(part 1 of 3)
# Autodesk Inventor assembly: FirstIntakes
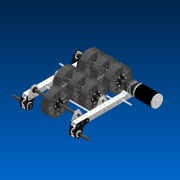
[picture p0: Inventor's stored thumbnail of the model, 180x180]
Saved by Autodesk Inventor 2022 (Build 260153000, 153)
## iProperties
Created: 2022-01-09
Part Number: FirstIntakes
Document SubType Name: Assembly
Designer: omard
Author: omard
## Documents named in this file (30)
- C:\Users\score_nygvs6w\OneDrive - Auburn University\BasketBall Shooting Robot\FirstIntakes.iam
- C:\Users\score_nygvs6w\OneDrive - Auburn University\BasketBall Shooting Robot\VEX Parts\VersaFrame Side Bearing Gusset (217-3553).ipt
- C:\Users\score_nygvs6w\OneDrive - Auburn University\BasketBall Shooting Robot\VEX Parts\13.75mm (1_2 ThunderHex ID) x 1.125 OD x 0.313 WD (Flanged Bearing) (217-4006).ipt
- C:\Users\score_nygvs6w\OneDrive - Auburn University\BasketBall Shooting Robot\VEX Parts\5 Straight Flex Wheel (60A) (217-6455).ipt
- C:\Users\score_nygvs6w\OneDrive - Auburn University\BasketBall Shooting Robot\VEX Parts\1_2” Hex Bore Plastic VersaHub v2 (217-8079).iam
- C:\Users\score_nygvs6w\OneDrive - Auburn University\BasketBall Shooting Robot\VEX Parts\24T x 9mm Wide Double Flange Aluminum Pulley (HTD 5mm, 1_2” Hex Bore) (217-3227).ipt
- C:\Users\score_nygvs6w\OneDrive - Auburn University\BasketBall Shooting Robot\VEX Parts\#8-32 x 2.000 Star Drive Screw (276-8015).ipt
- C:\Users\score_nygvs6w\OneDrive - Auburn University\BasketBall Shooting Robot\VEX Parts\#8-32 Nylock Nut (275-1027).ipt
- C:\Users\score_nygvs6w\OneDrive - Auburn University\BasketBall Shooting Robot\VEX Parts\1_4 Acetal Spacer - 1_2 Hex (217-2758).ipt
- C:\Users\score_nygvs6w\OneDrive - Auburn University\BasketBall Shooting Robot\VEX Parts\1_2 Acetal Spacer - 1_2 Hex (217-2758).ipt
- C:\Users\score_nygvs6w\OneDrive - Auburn University\BasketBall Shooting Robot\VEX Parts\80T x 9mm Wide Timing Belt (HTD 5mm)(217-3456).ipt
- C:\Users\score_nygvs6w\OneDrive - Auburn University\BasketBall Shooting Robot\VEX Parts\Clamping Shaft Collar - 1_2 Hex ID (217-2737).ipt
- C:\Users\score_nygvs6w\OneDrive - Auburn University\BasketBall Shooting Robot\VEX Parts\1_16 Acetal Spacer - 1_2 Hex (217-2758).ipt
- C:\Users\score_nygvs6w\OneDrive - Auburn University\BasketBall Shooting Robot\VEX Parts\#8-32 x 1.500 Star Drive Screw (276-4998).ipt
- C:\Users\score_nygvs6w\OneDrive - Auburn University\BasketBall Shooting Robot\Intake Joint Holder Using 1__16 Gray Tinted Polycarbonate Sheet (36 x 72) (217-6627).ipt
- C:\Users\score_nygvs6w\OneDrive - Auburn University\BasketBall Shooting Robot\VEX Parts\1.00 Standoff (275-1016).ipt
- C:\Users\score_nygvs6w\OneDrive - Auburn University\BasketBall Shooting Robot\VEX Parts\#8-32 x 0.500 Star Drive Screw (276-4992).ipt
- C:\Users\score_nygvs6w\OneDrive - Auburn University\BasketBall Shooting Robot\VEX Parts\1_8 Acetal Spacer - 1_2 Hex (217-2758).ipt
- C:\Users\score_nygvs6w\OneDrive - Auburn University\BasketBall Shooting Robot\VEX Parts\VersaPlanetary v2 One Stage Universal Output.iam
- C:\Users\score_nygvs6w\OneDrive - Auburn University\BasketBall Shooting Robot\VEX Parts\Special Cut\Intake VersaFrame VersaPlanetary Side Mount Modified (217-4239).ipt
- C:\Users\score_nygvs6w\OneDrive - Auburn University\BasketBall Shooting Robot\Intake Motor Holder Using 1__16 Gray Tinted Polycarbonate Sheet (36 x 72) (217-6627).ipt
- C:\Users\score_nygvs6w\OneDrive - Auburn University\BasketBall Shooting Robot\VEX Parts\Falcon 500, Powered by Talon FX (217-6515).iam
- C:\Users\score_nygvs6w\OneDrive - Auburn University\BasketBall Shooting Robot\VEX Parts\Special Cut\1 x 1 x 0.040 x 14 Intake Pre-Drilled VersaFrame Aluminum Tube Stock Cut Modified (217-3426).ipt
- C:\Users\score_nygvs6w\OneDrive - Auburn University\BasketBall Shooting Robot\VEX Parts\1_2 Hex x 0.201 x 10.5 ID ThunderHex Stock Cut (217-4017).ipt
- C:\Users\score_nygvs6w\OneDrive - Auburn University\BasketBall Shooting Robot\VEX Parts\1_2 Hex x 0.201 x 11 ID ThunderHex Stock Cut (217-4017).ipt
- C:\Users\score_nygvs6w\OneDrive - Auburn University\BasketBall Shooting Robot\VEX Parts\1_2 Hex x 0.201 x 4 ID ThunderHex Stock Cut (217-4017).ipt
- C:\Users\score_nygvs6w\OneDrive - Auburn University\BasketBall Shooting Robot\VEX Parts\5.00 Standoff  (275-1022).ipt
- C:\Users\score_nygvs6w\OneDrive - Auburn University\BasketBall Shooting Robot\VEX Parts\#8-32 x 1.000 Star Drive Coupler (276-4988).ipt
- C:\Users\score_nygvs6w\OneDrive - Auburn University\BasketBall Shooting Robot\VEX Parts\2.00 Standoff  (275-1018).ipt
- C:\Users\score_nygvs6w\OneDrive - Auburn University\BasketBall Shooting Robot\VEX Parts\CIM Motor (217-2000).ipt
## Components (233 placed, 29 different names)
1. VersaFrame Side Bearing Gusset (217-3553):2 — Mate:8, Mate:9, Mate:10, Mate:12, Mate:15, Mate:521, Mate:522
2. VersaFrame Side Bearing Gusset (217-3553):3 — Mate:1, Mate:2, Mate:3, Angle:1, Mate:13, Mate:14, Mate:523, Mate:524, Mate:525, Mate:636
3. 1 x 1 x 0.040 x 14 Intake Pre-Drilled VersaFrame Aluminum Tube Stock Cut Modified (217-3426):1 — Mate:1, Mate:2, Mate:3, Mate:8, Mate:9, Mate:10, Angle:1, Angle:2, Angle:3, Angle:20, Angle:133, Angle:134, Angle:135, Angle:136, Mate:494, Mate:495, Mate:496, Mate:497, Mate:498, Mate:499, Mate:500, Mate:501, Mate:505, Mate:506, Angle:203, Angle:204, Angle:205, Angle:206, Angle:207, Angle:208, Angle:209, Angle:210, Angle:211, Angle:212, Angle:213, Angle:214, Angle:215, Angle:216, Angle:217, Angle:218, Angle:258, Mate:630, Mate:631, Mate:632, Mate:633, Mate:634, Mate:635, Angle:262, Angle:263, Angle:264, Angle:265, Angle:266, Angle:268, Angle:274, Mate:699, Mate:700, Mate:701, Mate:702, Mate:703, Mate:704, Angle:279, Angle:280, Angle:281, Angle:282, Angle:283, Angle:284, Angle:285, Angle:286, Angle:287, Angle:288, Angle:289, Angle:290, Angle:291, Angle:292, Angle:293, Angle:294, Angle:295, Angle:296, Angle:297, Angle:298, Angle:299, Angle:300, Angle:301, Angle:302, Angle:303, Angle:304, Angle:305, Angle:306, Angle:307, Angle:308, Angle:309, Angle:310, Angle:311, Angle:312, Angle:313, Angle:314, Angle:317, Flush:563, Mate:742, Mate:743, Mate:744, Mate:745, Angle:330, Angle:331, Angle:335, Mate:752, Mate:753, Mate:754, Mate:757, Angle:337
4. 13.75mm (1_2 ThunderHex ID) x 1.125 OD x 0.313 WD (Flanged Bearing) (217-4006):1 — Mate:13, Mate:14, Mate:19, Angle:2, Mate:629, Mate:712, Flush:562
5. 13.75mm (1_2 ThunderHex ID) x 1.125 OD x 0.313 WD (Flanged Bearing) (217-4006):2 — Mate:12, Mate:15, Angle:3, Mate:448, Mate:526, Mate:713, Flush:561
6. 5 Straight Flex Wheel (60A) (217-6455):3 — Mate:19, Mate:22, Mate:23, Mate:28, Mate:31, Mate:34, Mate:37, Flush:2, Mate:455, Mate:558, Flush:560, Flush:14, Mate:610
7. 1_2” Hex Bore Plastic VersaHub v2 (217-8079):1 [sub-assembly] — Mate:31, Mate:34, Mate:37, Mate:90, Mate:93, Mate:94, Mate:95, Mate:96, Mate:97, Mate:98, Mate:99, Mate:100, Mate:101, Mate:102, Mate:103, Mate:104, Mate:117, Angle:35, Mate:118
8. 1_2” Hex Bore Plastic VersaHub v2 (217-8079):4 [sub-assembly] — Mate:22, Mate:23, Mate:28, Mate:111, Mate:112, Mate:113, Mate:114, Mate:115, Mate:116, Angle:23, Angle:24, Angle:25, Angle:26, Angle:27, Angle:28, Angle:185, Angle:186, Mate:467, Mate:468
9. 24T x 9mm Wide Double Flange Aluminum Pulley (HTD 5mm, 1_2” Hex Bore) (217-3227):3 — Mate:90, Angle:20, Angle:29, Angle:30, Angle:31, Angle:32, Angle:33, Angle:34, Angle:36, Mate:119, Flush:5, Mate:470, Mate:471, Mate:472, Angle:188
10. 1_4 Acetal Spacer - 1_2 Hex (217-2758):14 — Mate:117, Angle:35, Mate:118, Angle:36, Mate:119
11. 5 Straight Flex Wheel (60A) (217-6455):4 — Mate:406, Mate:407, Flush:1, Flush:2, Mate:448, Mate:477
12. 1_2” Hex Bore Plastic VersaHub v2 (217-8079):5 [sub-assembly]
13. 1_2” Hex Bore Plastic VersaHub v2 (217-8079):6 [sub-assembly] — Angle:219, Angle:221, Angle:222, Angle:223, Angle:224, Angle:220, Mate:547, Mate:548, Mate:550, Mate:551, Mate:552, Mate:553
14. 24T x 9mm Wide Double Flange Aluminum Pulley (HTD 5mm, 1_2” Hex Bore) (217-3227):5 — Mate:476
15. 1_4 Acetal Spacer - 1_2 Hex (217-2758):12 — Mate:463
16. 1_4 Acetal Spacer - 1_2 Hex (217-2758):11
17. 24T x 9mm Wide Double Flange Aluminum Pulley (HTD 5mm, 1_2” Hex Bore) (217-3227):6 — Angle:134, Mate:452, Flush:6
18. 5 Straight Flex Wheel (60A) (217-6455):5 — Mate:410, Mate:444, Flush:1
19. 1_2” Hex Bore Plastic VersaHub v2 (217-8079):7 [sub-assembly]
20. 1_2” Hex Bore Plastic VersaHub v2 (217-8079):8 [sub-assembly] — Angle:225, Angle:226, Angle:227, Angle:228, Angle:229, Angle:230, Mate:541, Mate:542, Mate:543, Mate:544, Mate:545, Mate:546
21. 1_2 Acetal Spacer - 1_2 Hex (217-2758):4 — Mate:487
22. 1_4 Acetal Spacer - 1_2 Hex (217-2758):8
23. 24T x 9mm Wide Double Flange Aluminum Pulley (HTD 5mm, 1_2” Hex Bore) (217-3227):8 — Angle:133, Angle:139, Angle:140, Tangent:1
24. 5 Straight Flex Wheel (60A) (217-6455):6 — Mate:410, Flush:4, Mate:456
25. 1_2” Hex Bore Plastic VersaHub v2 (217-8079):9 [sub-assembly]
26. 1_2” Hex Bore Plastic VersaHub v2 (217-8079):10 [sub-assembly] — Angle:232, Mate:556, Mate:557
27. 1_4 Acetal Spacer - 1_2 Hex (217-2758):9
28. 5 Straight Flex Wheel (60A) (217-6455):10 — Mate:406, Flush:11, Mate:477
29. 1_2” Hex Bore Plastic VersaHub v2 (217-8079):17 [sub-assembly] — Mate:346, Mate:347, Mate:462, Angle:181, Mate:474
30. 1_2” Hex Bore Plastic VersaHub v2 (217-8079):18 [sub-assembly] — Mate:475
31. 1_4 Acetal Spacer - 1_2 Hex (217-2758):13 — Angle:135, Mate:474, Mate:476
32. 5 Straight Flex Wheel (60A) (217-6455):11 — Mate:407, Flush:4, Mate:453, Mate:454
33. 1_2” Hex Bore Plastic VersaHub v2 (217-8079):19 [sub-assembly]
34. 1_2” Hex Bore Plastic VersaHub v2 (217-8079):20 [sub-assembly] — Angle:136, Mate:464, Mate:465, Angle:183
35. 1_4 Acetal Spacer - 1_2 Hex (217-2758):10 — Mate:452
36. 5 Straight Flex Wheel (60A) (217-6455):12 — Mate:444, Flush:11
37. 1_2” Hex Bore Plastic VersaHub v2 (217-8079):21 [sub-assembly] — Angle:231, Mate:554, Mate:555
38. 1_2” Hex Bore Plastic VersaHub v2 (217-8079):22 [sub-assembly] — Mate:446, Angle:132, Mate:447
39. 1_2 Acetal Spacer - 1_2 Hex (217-2758):3 — Mate:446, Angle:132, Mate:447, Angle:139, Angle:140, Mate:486, Angle:199
40. 80T x 9mm Wide Timing Belt (HTD 5mm)(217-3456):1 — Mate:454, Mate:456, Flush:6, Tangent:1
41. 80T x 9mm Wide Timing Belt (HTD 5mm)(217-3456):2 — Mate:453, Mate:455, Flush:5
42. Clamping Shaft Collar - 1_2 Hex ID (217-2737):1 — Angle:258, Mate:682, Mate:711
43. Clamping Shaft Collar - 1_2 Hex ID (217-2737):3 — Mate:464, Mate:465, Angle:183, Angle:233
44. Clamping Shaft Collar - 1_2 Hex ID (217-2737):4 — Mate:462, Angle:181, Angle:182, Mate:475
45. Clamping Shaft Collar - 1_2 Hex ID (217-2737):6 — Angle:182, Mate:463, Mate:526, Angle:315
46. Clamping Shaft Collar - 1_2 Hex ID (217-2737):7 — Mate:470, Angle:189, Mate:629, Angle:316
47. Clamping Shaft Collar - 1_2 Hex ID (217-2737):9 — Angle:185, Angle:186, Mate:467, Mate:468
48. Clamping Shaft Collar - 1_2 Hex ID (217-2737):10 — Mate:471, Mate:472, Angle:188, Angle:189
49. 1_16 Acetal Spacer - 1_2 Hex (217-2758):2 — Mate:486, Angle:199, Mate:487
50. Clamping Shaft Collar - 1_2 Hex ID (217-2737):12 — Angle:231, Mate:554, Mate:555, Mate:682
51. Clamping Shaft Collar - 1_2 Hex ID (217-2737):11 — Angle:232, Mate:556, Mate:557, Angle:233, Mate:673
52. VersaFrame Side Bearing Gusset (217-3553):4 — Mate:621
53. VersaFrame Side Bearing Gusset (217-3553):5
54. 1 x 1 x 0.040 x 14 Intake Pre-Drilled VersaFrame Aluminum Tube Stock Cut Modified (217-3426):2 — Angle:255, Angle:257, Mate:614, Mate:615, Mate:616, Mate:618, Mate:619, Mate:620, Angle:259, Angle:260, Angle:261, Angle:267, Angle:273, Mate:666, Mate:667, Mate:668, Mate:719, Angle:328, Angle:329, Mate:738, Mate:739, Mate:740, Mate:741, Mate:746, Mate:747, Mate:748, Mate:749, Angle:332, Angle:333, Mate:750, Mate:751, Angle:334, Mate:755, Mate:756, Angle:336
55. 13.75mm (1_2 ThunderHex ID) x 1.125 OD x 0.313 WD (Flanged Bearing) (217-4006):5 — Mate:628
56. 13.75mm (1_2 ThunderHex ID) x 1.125 OD x 0.313 WD (Flanged Bearing) (217-4006):6 — Mate:610, Mate:611, Mate:617
57. Clamping Shaft Collar - 1_2 Hex ID (217-2737):14 — Angle:257, Mate:628
58. Clamping Shaft Collar - 1_2 Hex ID (217-2737):15 — Mate:611, Angle:255, Mate:617
59. Intake Joint Holder Using 1__16 Gray Tinted Polycarbonate Sheet (36 x 72) (217-6627):1 — Mate:584, Mate:585, Mate:583, Mate:614, Mate:615, Mate:616, Mate:622, Mate:623, Mate:626, Mate:627, Mate:650, Mate:651
60. Intake Joint Holder Using 1__16 Gray Tinted Polycarbonate Sheet (36 x 72) (217-6627):2 — Mate:618, Mate:619, Mate:620, Mate:621, Mate:625, Mate:652, Mate:653
61. Intake Joint Holder Using 1__16 Gray Tinted Polycarbonate Sheet (36 x 72) (217-6627):3 — Mate:630, Mate:631, Mate:632, Mate:636, Mate:641, Mate:643, Mate:645, Mate:647, Mate:649
62. Intake Joint Holder Using 1__16 Gray Tinted Polycarbonate Sheet (36 x 72) (217-6627):4 — Mate:633, Mate:634, Mate:635, Mate:637, Mate:638, Mate:639, Mate:642, Mate:644, Mate:646, Mate:648
63. 1.00 Standoff (275-1016):1 — Mate:622, Mate:623, Mate:624, Angle:261
64. 1.00 Standoff (275-1016):2 — Mate:643, Angle:264
65. 13.75mm (1_2 ThunderHex ID) x 1.125 OD x 0.313 WD (Flanged Bearing) (217-4006):7 — Mate:646, Mate:648, Angle:265, Mate:664, Mate:665, Mate:722, Mate:723
66. 13.75mm (1_2 ThunderHex ID) x 1.125 OD x 0.313 WD (Flanged Bearing) (217-4006):8 — Mate:652, Angle:268, Mate:653, Mate:724, Mate:725
67. 13.75mm (1_2 ThunderHex ID) x 1.125 OD x 0.313 WD (Flanged Bearing) (217-4006):9 — Mate:650, Mate:651, Angle:267, Mate:662, Mate:663, Mate:720, Mate:721
68. 13.75mm (1_2 ThunderHex ID) x 1.125 OD x 0.313 WD (Flanged Bearing) (217-4006):10 — Mate:647, Mate:649, Angle:266, Mate:726, Mate:727
69. 1_2 Acetal Spacer - 1_2 Hex (217-2758):5 — Mate:662, Mate:663, Angle:273, Angle:318
70. 1_4 Acetal Spacer - 1_2 Hex (217-2758):15
71. 1_8 Acetal Spacer - 1_2 Hex (217-2758):1 — Angle:320
72. 1_2 Acetal Spacer - 1_2 Hex (217-2758):6 — Angle:274, Angle:319, Angle:321
73. 1_4 Acetal Spacer - 1_2 Hex (217-2758):16
74. 1_8 Acetal Spacer - 1_2 Hex (217-2758):2 — Mate:664, Mate:665
75. Intake VersaFrame VersaPlanetary Side Mount Modified (217-4239):1 — Mate:666, Mate:667, Mate:668, Mate:669, Mate:670, Mate:671, Mate:590, Mate:674, Mate:675, Mate:676, Mate:677, Mate:678, Mate:679, Mate:680, Mate:681, Angle:275, Angle:276
76. VersaPlanetary v2 One Stage Universal Output:1 [sub-assembly] — Mate:669, Mate:670, Mate:671, Mate:673, Mate:714, Mate:715, Mate:716, Mate:718, Mate:758, Mate:759, Mate:760
77. Intake Motor Holder Using 1__16 Gray Tinted Polycarbonate Sheet (36 x 72) (217-6627):1 — Mate:701, Mate:702, Mate:703, Mate:708, Mate:709, Mate:710
78. Intake Motor Holder Using 1__16 Gray Tinted Polycarbonate Sheet (36 x 72) (217-6627):2 — Mate:699, Mate:700, Mate:704, Mate:705, Mate:706, Mate:707
79. 1.00 Standoff (275-1016):3 — Angle:279
80. 13.75mm (1_2 ThunderHex ID) x 1.125 OD x 0.313 WD (Flanged Bearing) (217-4006):11 — Angle:282, Mate:717
81. 13.75mm (1_2 ThunderHex ID) x 1.125 OD x 0.313 WD (Flanged Bearing) (217-4006):12 — Mate:711, Angle:283
82. 1_2 Acetal Spacer - 1_2 Hex (217-2758):7 — Angle:284
83. 1_4 Acetal Spacer - 1_2 Hex (217-2758):17
84. 1_8 Acetal Spacer - 1_2 Hex (217-2758):3
85. 1_2 Hex x 0.201 x 10.5 ID ThunderHex Stock Cut (217-4017):1 — Mate:712, Angle:316, Flush:562
86. 1_2 Hex x 0.201 x 10.5 ID ThunderHex Stock Cut (217-4017):2 — Mate:713, Angle:315, Flush:561
87. Falcon 500, Powered by Talon FX (217-6515):1 [sub-assembly] — Mate:714, Mate:715, Mate:716
88. 1_2 Hex x 0.201 x 11 ID ThunderHex Stock Cut (217-4017):1 — Mate:717, Angle:317, Mate:718
89. 1_2 Acetal Spacer - 1_2 Hex (217-2758):8 — Mate:720, Mate:721, Angle:318, Angle:322
90. 1_2 Acetal Spacer - 1_2 Hex (217-2758):9 — Angle:319, Mate:722, Mate:723
91. Clamping Shaft Collar - 1_2 Hex ID (217-2737):16 — Mate:724, Angle:320, Mate:725, Flush:565, Mate:728
92. Clamping Shaft Collar - 1_2 Hex ID (217-2737):17 — Angle:321, Mate:726, Mate:727, Angle:323, Flush:564, Mate:729
93. 1_2 Hex x 0.201 x 4 ID ThunderHex Stock Cut (217-4017):1 — Angle:322, Flush:565, Mate:728
94. 1_2 Hex x 0.201 x 4 ID ThunderHex Stock Cut (217-4017):2 — Angle:323, Flush:564, Mate:729
95. 5.00 Standoff  (275-1022):1 — Mate:730, Angle:324, Mate:732, Mate:733, Angle:329, Mate:738, Mate:740
96. 5.00 Standoff  (275-1022):2 — Mate:731, Angle:324, Mate:733, Angle:325
97. 5.00 Standoff  (275-1022):3 — Angle:328, Mate:739, Mate:741
98. 5.00 Standoff  (275-1022):4 — Angle:327
99. 2.00 Standoff  (275-1018):1 — Mate:750, Mate:751, Angle:334
100. 2.00 Standoff  (275-1018):2 — Angle:335, Mate:752, Mate:753
101. CIM Motor (217-2000):1 — Mate:758, Mate:759, Mate:760
102. #8-32 x 1.500 Star Drive Screw (276-4998):21 — Mate:755, Mate:756, Angle:336
103. #8-32 x 1.500 Star Drive Screw (276-4998):22 — Mate:754, Mate:757, Angle:337
104. #8-32 x 1.500 Star Drive Screw (276-4998):20 — Mate:743, Mate:745, Angle:330
105. #8-32 x 1.500 Star Drive Screw (276-4998):19 — Mate:742, Mate:744, Angle:331
106. #8-32 x 1.500 Star Drive Screw (276-4998):18 — Mate:746, Mate:749, Angle:332
107. #8-32 x 1.500 Star Drive Screw (276-4998):17 — Mate:747, Mate:748, Angle:333
108. #8-32 x 1.000 Star Drive Coupler (276-4988):1 — Mate:730, Mate:731, Mate:732, Angle:325
109. #8-32 x 1.000 Star Drive Coupler (276-4988):2 — Angle:327
110. #8-32 x 0.500 Star Drive Screw (276-4992):8 — Angle:281
111. #8-32 x 0.500 Star Drive Screw (276-4992):7 — Angle:280
112. #8-32 x 0.500 Star Drive Screw (276-4992):6 — Mate:678, Mate:681, Angle:276
113. #8-32 x 0.500 Star Drive Screw (276-4992):5 — Mate:679, Mate:680, Angle:275
114. #8-32 x 0.500 Star Drive Screw (276-4992):3 — Mate:642, Mate:644, Angle:263
115. #8-32 x 0.500 Star Drive Screw (276-4992):4 — Mate:641, Mate:645, Angle:262
116. #8-32 x 0.500 Star Drive Screw (276-4992):1 — Mate:624, Mate:625, Angle:260
117. #8-32 x 0.500 Star Drive Screw (276-4992):2 — Mate:626, Mate:627, Angle:259
118. #8-32 x 1.500 Star Drive Screw (276-4998):9 — Mate:590
119. #8-32 x 1.500 Star Drive Screw (276-4998):10
120. #8-32 x 1.500 Star Drive Screw (276-4998):11 — Mate:674
121. #8-32 x 1.500 Star Drive Screw (276-4998):12
122. #8-32 x 1.500 Star Drive Screw (276-4998):13
123. #8-32 x 1.500 Star Drive Screw (276-4998):14 — Mate:584
124. #8-32 x 1.500 Star Drive Screw (276-4998):15 — Mate:585
125. #8-32 x 1.500 Star Drive Screw (276-4998):16 — Mate:583
126. #8-32 Nylock Nut (275-1027):81
127. #8-32 Nylock Nut (275-1027):82
128. #8-32 Nylock Nut (275-1027):83 — Mate:676
129. #8-32 Nylock Nut (275-1027):84 — Mate:677
130. #8-32 Nylock Nut (275-1027):85 — Mate:675
131. #8-32 Nylock Nut (275-1027):86
132. #8-32 Nylock Nut (275-1027):87
133. #8-32 Nylock Nut (275-1027):88
134. #8-32 Nylock Nut (275-1027):69 — Mate:529, Angle:224, Mate:552
135. #8-32 Nylock Nut (275-1027):70 — Mate:530, Angle:219, Mate:553
136. #8-32 Nylock Nut (275-1027):71 — Mate:531, Angle:220, Mate:548
137. #8-32 Nylock Nut (275-1027):72 — Mate:532, Angle:221, Mate:550
138. #8-32 Nylock Nut (275-1027):73 — Mate:533, Angle:222, Mate:547
139. #8-32 Nylock Nut (275-1027):74 — Mate:535, Angle:228, Mate:541
140. #8-32 Nylock Nut (275-1027):75 — Mate:536, Angle:227, Mate:543
141. #8-32 Nylock Nut (275-1027):76 — Mate:538, Angle:226, Mate:545
142. #8-32 Nylock Nut (275-1027):77 — Mate:539, Angle:229, Mate:544
143. #8-32 Nylock Nut (275-1027):78 — Mate:540, Angle:225, Mate:546
144. #8-32 Nylock Nut (275-1027):79 — Mate:537, Angle:230, Mate:542
145. #8-32 Nylock Nut (275-1027):80 — Mate:534, Angle:223, Mate:551
146. #8-32 x 1.500 Star Drive Screw (276-4998):1 — Mate:494, Mate:510, Angle:211, Mate:637
147. #8-32 x 1.500 Star Drive Screw (276-4998):2 — Mate:495, Mate:511, Angle:218, Mate:638
148. #8-32 x 1.500 Star Drive Screw (276-4998):3 — Mate:496, Mate:512, Angle:217, Mate:639
149. #8-32 x 1.500 Star Drive Screw (276-4998):4 — Mate:497, Mate:505, Mate:514, Angle:216
150. #8-32 x 1.500 Star Drive Screw (276-4998):5 — Mate:498, Mate:506, Mate:513, Angle:215
151. #8-32 x 1.500 Star Drive Screw (276-4998):6 — Mate:500, Mate:516, Angle:214, Mate:706
152. #8-32 x 1.500 Star Drive Screw (276-4998):7 — Mate:499, Mate:517, Angle:213, Mate:707
153. #8-32 x 1.500 Star Drive Screw (276-4998):8 — Mate:501, Mate:515, Angle:212, Mate:705
154. #8-32 Nylock Nut (275-1027):61 — Mate:514, Mate:521, Angle:206
155. #8-32 Nylock Nut (275-1027):62 — Mate:513, Mate:522, Angle:207
156. #8-32 Nylock Nut (275-1027):63 — Mate:511, Mate:524, Angle:209
157. #8-32 Nylock Nut (275-1027):64 — Mate:512, Mate:525, Angle:208
158. #8-32 Nylock Nut (275-1027):65 — Mate:510, Mate:523, Angle:210
159. #8-32 Nylock Nut (275-1027):66 — Mate:515, Angle:203, Mate:708
160. #8-32 Nylock Nut (275-1027):67 — Mate:516, Angle:204, Mate:709
161. #8-32 Nylock Nut (275-1027):68 — Mate:517, Angle:205, Mate:710
162. #8-32 x 2.000 Star Drive Screw (276-8015):49 — Angle:314
163. #8-32 x 2.000 Star Drive Screw (276-8015):50 — Angle:313
164. #8-32 x 2.000 Star Drive Screw (276-8015):51 — Angle:312
165. #8-32 x 2.000 Star Drive Screw (276-8015):52 — Angle:311
166. #8-32 x 2.000 Star Drive Screw (276-8015):53 — Angle:310
167. #8-32 x 2.000 Star Drive Screw (276-8015):54 — Angle:309
168. #8-32 Nylock Nut (275-1027):49
169. #8-32 Nylock Nut (275-1027):50
170. #8-32 Nylock Nut (275-1027):51
171. #8-32 Nylock Nut (275-1027):52
172. #8-32 Nylock Nut (275-1027):53
173. #8-32 Nylock Nut (275-1027):54
174. #8-32 x 2.000 Star Drive Screw (276-8015):55 — Angle:308
175. #8-32 x 2.000 Star Drive Screw (276-8015):56 — Angle:307
176. #8-32 x 2.000 Star Drive Screw (276-8015):57 — Angle:306
177. #8-32 x 2.000 Star Drive Screw (276-8015):58 — Angle:305
178. #8-32 x 2.000 Star Drive Screw (276-8015):59 — Angle:304
179. #8-32 x 2.000 Star Drive Screw (276-8015):60 — Angle:303
180. #8-32 Nylock Nut (275-1027):55
181. #8-32 Nylock Nut (275-1027):56
182. #8-32 Nylock Nut (275-1027):57
183. #8-32 Nylock Nut (275-1027):58
184. #8-32 Nylock Nut (275-1027):59
185. #8-32 Nylock Nut (275-1027):60
186. #8-32 x 2.000 Star Drive Screw (276-8015):43 — Mate:347, Angle:302
187. #8-32 x 2.000 Star Drive Screw (276-8015):44 — Angle:301
188. #8-32 x 2.000 Star Drive Screw (276-8015):45 — Angle:300
189. #8-32 x 2.000 Star Drive Screw (276-8015):46 — Angle:299
190. #8-32 x 2.000 Star Drive Screw (276-8015):47 — Angle:298
191. #8-32 x 2.000 Star Drive Screw (276-8015):48 — Mate:346, Angle:297
192. #8-32 Nylock Nut (275-1027):43
193. #8-32 Nylock Nut (275-1027):44
194. #8-32 Nylock Nut (275-1027):45
195. #8-32 Nylock Nut (275-1027):46
196. #8-32 Nylock Nut (275-1027):47
197. #8-32 Nylock Nut (275-1027):48
198. #8-32 x 2.000 Star Drive Screw (276-8015):19 — Angle:296
199. #8-32 x 2.000 Star Drive Screw (276-8015):20 — Angle:295
200. #8-32 x 2.000 Star Drive Screw (276-8015):21 — Angle:294
201. #8-32 x 2.000 Star Drive Screw (276-8015):22 — Angle:293
202. #8-32 x 2.000 Star Drive Screw (276-8015):23 — Angle:292
203. #8-32 x 2.000 Star Drive Screw (276-8015):24 — Angle:291
204. #8-32 Nylock Nut (275-1027):19
205. #8-32 Nylock Nut (275-1027):20
206. #8-32 Nylock Nut (275-1027):21
207. #8-32 Nylock Nut (275-1027):22
208. #8-32 Nylock Nut (275-1027):23
209. #8-32 Nylock Nut (275-1027):24
210. #8-32 x 2.000 Star Drive Screw (276-8015):69 — Mate:537, Angle:290
211. #8-32 x 2.000 Star Drive Screw (276-8015):68 — Mate:536, Angle:289
212. #8-32 x 2.000 Star Drive Screw (276-8015):72 — Mate:540, Angle:288
213. #8-32 x 2.000 Star Drive Screw (276-8015):71 — Mate:538, Angle:287
214. #8-32 x 2.000 Star Drive Screw (276-8015):67 — Mate:535, Angle:286
215. #8-32 x 2.000 Star Drive Screw (276-8015):70 — Mate:539, Angle:285
216. #8-32 x 2.000 Star Drive Screw (276-8015):66 — Mate:531
217. #8-32 x 2.000 Star Drive Screw (276-8015):65 — Mate:533
218. #8-32 x 2.000 Star Drive Screw (276-8015):61 — Mate:529
219. #8-32 x 2.000 Star Drive Screw (276-8015):62 — Mate:534
220. #8-32 x 2.000 Star Drive Screw (276-8015):64 — Mate:532
221. #8-32 x 2.000 Star Drive Screw (276-8015):63 — Mate:530
222. #8-32 x 2.000 Star Drive Screw (276-8015):1 — Mate:96, Mate:103, Mate:107, Angle:29
223. #8-32 x 2.000 Star Drive Screw (276-8015):2 — Mate:97, Mate:99, Mate:109, Angle:34
224. #8-32 x 2.000 Star Drive Screw (276-8015):3 — Mate:93, Mate:101, Mate:105, Angle:33
225. #8-32 x 2.000 Star Drive Screw (276-8015):4 — Mate:94, Mate:100, Mate:110, Angle:32
226. #8-32 x 2.000 Star Drive Screw (276-8015):5 — Mate:98, Mate:102, Mate:108, Angle:31
227. #8-32 x 2.000 Star Drive Screw (276-8015):6 — Mate:95, Mate:104, Mate:106, Angle:30
228. #8-32 Nylock Nut (275-1027):1 — Mate:106, Mate:116, Angle:24
229. #8-32 Nylock Nut (275-1027):2 — Mate:108, Mate:114, Angle:26
230. #8-32 Nylock Nut (275-1027):3 — Mate:110, Mate:112, Angle:28
231. #8-32 Nylock Nut (275-1027):4 — Mate:109, Mate:113, Angle:27
232. #8-32 Nylock Nut (275-1027):5 — Mate:107, Mate:115, Angle:25
233. #8-32 Nylock Nut (275-1027):6 — Mate:105, Mate:111, Angle:23
## Relationships (704: Mate 486, Angle 204, Flush 13, Tangent 1)
- Mate:1: VersaFrame Side Bearing Gusset (217-3553):3 ↔ 1 x 1 x 0.040 x 14 Intake Pre-Drilled VersaFrame Aluminum Tube Stock Cut Modified (217-3426):1
- Mate:2: VersaFrame Side Bearing Gusset (217-3553):3 ↔ 1 x 1 x 0.040 x 14 Intake Pre-Drilled VersaFrame Aluminum Tube Stock Cut Modified (217-3426):1
- Mate:3: VersaFrame Side Bearing Gusset (217-3553):3 ↔ 1 x 1 x 0.040 x 14 Intake Pre-Drilled VersaFrame Aluminum Tube Stock Cut Modified (217-3426):1
- Mate:8: VersaFrame Side Bearing Gusset (217-3553):2 ↔ 1 x 1 x 0.040 x 14 Intake Pre-Drilled VersaFrame Aluminum Tube Stock Cut Modified (217-3426):1
- Mate:9: VersaFrame Side Bearing Gusset (217-3553):2 ↔ 1 x 1 x 0.040 x 14 Intake Pre-Drilled VersaFrame Aluminum Tube Stock Cut Modified (217-3426):1
- Mate:10: VersaFrame Side Bearing Gusset (217-3553):2 ↔ 1 x 1 x 0.040 x 14 Intake Pre-Drilled VersaFrame Aluminum Tube Stock Cut Modified (217-3426):1
- Angle:1 (0 deg): VersaFrame Side Bearing Gusset (217-3553):3 ↔ 1 x 1 x 0.040 x 14 Intake Pre-Drilled VersaFrame Aluminum Tube Stock Cut Modified (217-3426):1
- Mate:12: VersaFrame Side Bearing Gusset (217-3553):2 ↔ 13.75mm (1_2 ThunderHex ID) x 1.125 OD x 0.313 WD (Flanged Bearing) (217-4006):2
- Mate:13: VersaFrame Side Bearing Gusset (217-3553):3 ↔ 13.75mm (1_2 ThunderHex ID) x 1.125 OD x 0.313 WD (Flanged Bearing) (217-4006):1
- Mate:14: VersaFrame Side Bearing Gusset (217-3553):3 ↔ 13.75mm (1_2 ThunderHex ID) x 1.125 OD x 0.313 WD (Flanged Bearing) (217-4006):1
- Mate:15: VersaFrame Side Bearing Gusset (217-3553):2 ↔ 13.75mm (1_2 ThunderHex ID) x 1.125 OD x 0.313 WD (Flanged Bearing) (217-4006):2
- Mate:19: 13.75mm (1_2 ThunderHex ID) x 1.125 OD x 0.313 WD (Flanged Bearing) (217-4006):1 ↔ 5 Straight Flex Wheel (60A) (217-6455):3
- Angle:2 (0 deg): 1 x 1 x 0.040 x 14 Intake Pre-Drilled VersaFrame Aluminum Tube Stock Cut Modified (217-3426):1 ↔ 13.75mm (1_2 ThunderHex ID) x 1.125 OD x 0.313 WD (Flanged Bearing) (217-4006):1
- Angle:3 (0 deg): 1 x 1 x 0.040 x 14 Intake Pre-Drilled VersaFrame Aluminum Tube Stock Cut Modified (217-3426):1 ↔ 13.75mm (1_2 ThunderHex ID) x 1.125 OD x 0.313 WD (Flanged Bearing) (217-4006):2
- Mate:22: 5 Straight Flex Wheel (60A) (217-6455):3 ↔ 1_2” Hex Bore Plastic VersaHub v2 (217-8079):4
- Mate:23: 5 Straight Flex Wheel (60A) (217-6455):3 ↔ 1_2” Hex Bore Plastic VersaHub v2 (217-8079):4
- Mate:28: 5 Straight Flex Wheel (60A) (217-6455):3 ↔ 1_2” Hex Bore Plastic VersaHub v2 (217-8079):4
- Mate:31: 5 Straight Flex Wheel (60A) (217-6455):3 ↔ 1_2” Hex Bore Plastic VersaHub v2 (217-8079):1
- Mate:34: 5 Straight Flex Wheel (60A) (217-6455):3 ↔ 1_2” Hex Bore Plastic VersaHub v2 (217-8079):1
- Mate:37: 5 Straight Flex Wheel (60A) (217-6455):3 ↔ 1_2” Hex Bore Plastic VersaHub v2 (217-8079):1
- Mate:90: 1_2” Hex Bore Plastic VersaHub v2 (217-8079):1 ↔ 24T x 9mm Wide Double Flange Aluminum Pulley (HTD 5mm, 1_2” Hex Bore) (217-3227):3
- Angle:20 (0 deg): 1 x 1 x 0.040 x 14 Intake Pre-Drilled VersaFrame Aluminum Tube Stock Cut Modified (217-3426):1 ↔ 24T x 9mm Wide Double Flange Aluminum Pulley (HTD 5mm, 1_2” Hex Bore) (217-3227):3
- Mate:93: 1_2” Hex Bore Plastic VersaHub v2 (217-8079):1 ↔ #8-32 x 2.000 Star Drive Screw (276-8015):3
- Mate:94: 1_2” Hex Bore Plastic VersaHub v2 (217-8079):1 ↔ #8-32 x 2.000 Star Drive Screw (276-8015):4
- Mate:95: 1_2” Hex Bore Plastic VersaHub v2 (217-8079):1 ↔ #8-32 x 2.000 Star Drive Screw (276-8015):6
- Mate:96: 1_2” Hex Bore Plastic VersaHub v2 (217-8079):1 ↔ #8-32 x 2.000 Star Drive Screw (276-8015):1
- Mate:97: 1_2” Hex Bore Plastic VersaHub v2 (217-8079):1 ↔ #8-32 x 2.000 Star Drive Screw (276-8015):2
- Mate:98: 1_2” Hex Bore Plastic VersaHub v2 (217-8079):1 ↔ #8-32 x 2.000 Star Drive Screw (276-8015):5
- Mate:99: 1_2” Hex Bore Plastic VersaHub v2 (217-8079):1 ↔ #8-32 x 2.000 Star Drive Screw (276-8015):2
- Mate:100: 1_2” Hex Bore Plastic VersaHub v2 (217-8079):1 ↔ #8-32 x 2.000 Star Drive Screw (276-8015):4
- Mate:101: 1_2” Hex Bore Plastic VersaHub v2 (217-8079):1 ↔ #8-32 x 2.000 Star Drive Screw (276-8015):3
- Mate:102: 1_2” Hex Bore Plastic VersaHub v2 (217-8079):1 ↔ #8-32 x 2.000 Star Drive Screw (276-8015):5
- Mate:103: 1_2” Hex Bore Plastic VersaHub v2 (217-8079):1 ↔ #8-32 x 2.000 Star Drive Screw (276-8015):1
- Mate:104: 1_2” Hex Bore Plastic VersaHub v2 (217-8079):1 ↔ #8-32 x 2.000 Star Drive Screw (276-8015):6
- Mate:105: #8-32 x 2.000 Star Drive Screw (276-8015):3 ↔ #8-32 Nylock Nut (275-1027):6
- Mate:106: #8-32 x 2.000 Star Drive Screw (276-8015):6 ↔ #8-32 Nylock Nut (275-1027):1
- Mate:107: #8-32 x 2.000 Star Drive Screw (276-8015):1 ↔ #8-32 Nylock Nut (275-1027):5
- Mate:108: #8-32 x 2.000 Star Drive Screw (276-8015):5 ↔ #8-32 Nylock Nut (275-1027):2
- Mate:109: #8-32 x 2.000 Star Drive Screw (276-8015):2 ↔ #8-32 Nylock Nut (275-1027):4
- Mate:110: #8-32 x 2.000 Star Drive Screw (276-8015):4 ↔ #8-32 Nylock Nut (275-1027):3
- Mate:111: 1_2” Hex Bore Plastic VersaHub v2 (217-8079):4 ↔ #8-32 Nylock Nut (275-1027):6
- Mate:112: 1_2” Hex Bore Plastic VersaHub v2 (217-8079):4 ↔ #8-32 Nylock Nut (275-1027):3
- Mate:113: 1_2” Hex Bore Plastic VersaHub v2 (217-8079):4 ↔ #8-32 Nylock Nut (275-1027):4
- Mate:114: 1_2” Hex Bore Plastic VersaHub v2 (217-8079):4 ↔ #8-32 Nylock Nut (275-1027):2
- Mate:115: 1_2” Hex Bore Plastic VersaHub v2 (217-8079):4 ↔ #8-32 Nylock Nut (275-1027):5
- Mate:116: 1_2” Hex Bore Plastic VersaHub v2 (217-8079):4 ↔ #8-32 Nylock Nut (275-1027):1
- Angle:23 (0 deg): 1_2” Hex Bore Plastic VersaHub v2 (217-8079):4 ↔ #8-32 Nylock Nut (275-1027):6
- Angle:24 (0 deg): 1_2” Hex Bore Plastic VersaHub v2 (217-8079):4 ↔ #8-32 Nylock Nut (275-1027):1
- Angle:25 (0 deg): 1_2” Hex Bore Plastic VersaHub v2 (217-8079):4 ↔ #8-32 Nylock Nut (275-1027):5
- Angle:26 (0 deg): 1_2” Hex Bore Plastic VersaHub v2 (217-8079):4 ↔ #8-32 Nylock Nut (275-1027):2
- Angle:27 (0 deg): 1_2” Hex Bore Plastic VersaHub v2 (217-8079):4 ↔ #8-32 Nylock Nut (275-1027):4
- Angle:28 (0 deg): 1_2” Hex Bore Plastic VersaHub v2 (217-8079):4 ↔ #8-32 Nylock Nut (275-1027):3
- Angle:29 (0 deg): 24T x 9mm Wide Double Flange Aluminum Pulley (HTD 5mm, 1_2” Hex Bore) (217-3227):3 ↔ #8-32 x 2.000 Star Drive Screw (276-8015):1
- Angle:30 (0 deg): 24T x 9mm Wide Double Flange Aluminum Pulley (HTD 5mm, 1_2” Hex Bore) (217-3227):3 ↔ #8-32 x 2.000 Star Drive Screw (276-8015):6
- Angle:31 (0 deg): 24T x 9mm Wide Double Flange Aluminum Pulley (HTD 5mm, 1_2” Hex Bore) (217-3227):3 ↔ #8-32 x 2.000 Star Drive Screw (276-8015):5
- Angle:32 (0 deg): 24T x 9mm Wide Double Flange Aluminum Pulley (HTD 5mm, 1_2” Hex Bore) (217-3227):3 ↔ #8-32 x 2.000 Star Drive Screw (276-8015):4
- Angle:33 (0 deg): 24T x 9mm Wide Double Flange Aluminum Pulley (HTD 5mm, 1_2” Hex Bore) (217-3227):3 ↔ #8-32 x 2.000 Star Drive Screw (276-8015):3
- Angle:34 (0 deg): 24T x 9mm Wide Double Flange Aluminum Pulley (HTD 5mm, 1_2” Hex Bore) (217-3227):3 ↔ #8-32 x 2.000 Star Drive Screw (276-8015):2
- Mate:117: 1_2” Hex Bore Plastic VersaHub v2 (217-8079):1 ↔ 1_4 Acetal Spacer - 1_2 Hex (217-2758):14
- Angle:35 (0 deg): 1_2” Hex Bore Plastic VersaHub v2 (217-8079):1 ↔ 1_4 Acetal Spacer - 1_2 Hex (217-2758):14
- Mate:118: 1_2” Hex Bore Plastic VersaHub v2 (217-8079):1 ↔ 1_4 Acetal Spacer - 1_2 Hex (217-2758):14
- Angle:36 (0 deg): 24T x 9mm Wide Double Flange Aluminum Pulley (HTD 5mm, 1_2” Hex Bore) (217-3227):3 ↔ 1_4 Acetal Spacer - 1_2 Hex (217-2758):14
- Mate:119: 24T x 9mm Wide Double Flange Aluminum Pulley (HTD 5mm, 1_2” Hex Bore) (217-3227):3 ↔ 1_4 Acetal Spacer - 1_2 Hex (217-2758):14
- [Mate]: 5 Straight Flex Wheel (60A) (217-6455):4 ↔ 1_2” Hex Bore Plastic VersaHub v2 (217-8079):6
- [Mate]: 5 Straight Flex Wheel (60A) (217-6455):4 ↔ 1_2” Hex Bore Plastic VersaHub v2 (217-8079):6
- [Mate]: 5 Straight Flex Wheel (60A) (217-6455):4 ↔ 1_2” Hex Bore Plastic VersaHub v2 (217-8079):6
- [Mate]: 5 Straight Flex Wheel (60A) (217-6455):4 ↔ 1_2” Hex Bore Plastic VersaHub v2 (217-8079):5
- [Mate]: 5 Straight Flex Wheel (60A) (217-6455):4 ↔ 1_2” Hex Bore Plastic VersaHub v2 (217-8079):5
- [Mate]: 5 Straight Flex Wheel (60A) (217-6455):4 ↔ 1_2” Hex Bore Plastic VersaHub v2 (217-8079):5
- [Mate]: 1_2” Hex Bore Plastic VersaHub v2 (217-8079):5 ↔ 24T x 9mm Wide Double Flange Aluminum Pulley (HTD 5mm, 1_2” Hex Bore) (217-3227):5
- [Mate]: 1_2” Hex Bore Plastic VersaHub v2 (217-8079):5 ↔ #8-32 x 2.000 Star Drive Screw (276-8015):61
- [Mate]: 1_2” Hex Bore Plastic VersaHub v2 (217-8079):5 ↔ #8-32 x 2.000 Star Drive Screw (276-8015):62
- [Mate]: 1_2” Hex Bore Plastic VersaHub v2 (217-8079):5 ↔ #8-32 x 2.000 Star Drive Screw (276-8015):63
- [Mate]: 1_2” Hex Bore Plastic VersaHub v2 (217-8079):5 ↔ #8-32 x 2.000 Star Drive Screw (276-8015):66
- [Mate]: 1_2” Hex Bore Plastic VersaHub v2 (217-8079):5 ↔ #8-32 x 2.000 Star Drive Screw (276-8015):65
- [Mate]: 1_2” Hex Bore Plastic VersaHub v2 (217-8079):5 ↔ #8-32 x 2.000 Star Drive Screw (276-8015):64
- [Mate]: 1_2” Hex Bore Plastic VersaHub v2 (217-8079):5 ↔ #8-32 x 2.000 Star Drive Screw (276-8015):65
- [Mate]: 1_2” Hex Bore Plastic VersaHub v2 (217-8079):5 ↔ #8-32 x 2.000 Star Drive Screw (276-8015):62
- [Mate]: 1_2” Hex Bore Plastic VersaHub v2 (217-8079):5 ↔ #8-32 x 2.000 Star Drive Screw (276-8015):61
- [Mate]: 1_2” Hex Bore Plastic VersaHub v2 (217-8079):5 ↔ #8-32 x 2.000 Star Drive Screw (276-8015):64
- [Mate]: 1_2” Hex Bore Plastic VersaHub v2 (217-8079):5 ↔ #8-32 x 2.000 Star Drive Screw (276-8015):66
- [Mate]: 1_2” Hex Bore Plastic VersaHub v2 (217-8079):5 ↔ #8-32 x 2.000 Star Drive Screw (276-8015):63
- [Angle] (0 deg): 24T x 9mm Wide Double Flange Aluminum Pulley (HTD 5mm, 1_2” Hex Bore) (217-3227):5 ↔ #8-32 x 2.000 Star Drive Screw (276-8015):66
- [Angle] (0 deg): 24T x 9mm Wide Double Flange Aluminum Pulley (HTD 5mm, 1_2” Hex Bore) (217-3227):5 ↔ #8-32 x 2.000 Star Drive Screw (276-8015):63
- [Angle] (0 deg): 24T x 9mm Wide Double Flange Aluminum Pulley (HTD 5mm, 1_2” Hex Bore) (217-3227):5 ↔ #8-32 x 2.000 Star Drive Screw (276-8015):64
- [Angle] (0 deg): 24T x 9mm Wide Double Flange Aluminum Pulley (HTD 5mm, 1_2” Hex Bore) (217-3227):5 ↔ #8-32 x 2.000 Star Drive Screw (276-8015):62
- [Angle] (0 deg): 24T x 9mm Wide Double Flange Aluminum Pulley (HTD 5mm, 1_2” Hex Bore) (217-3227):5 ↔ #8-32 x 2.000 Star Drive Screw (276-8015):61
- [Angle] (0 deg): 24T x 9mm Wide Double Flange Aluminum Pulley (HTD 5mm, 1_2” Hex Bore) (217-3227):5 ↔ #8-32 x 2.000 Star Drive Screw (276-8015):65
- [Mate]: 1_2” Hex Bore Plastic VersaHub v2 (217-8079):5 ↔ 1_4 Acetal Spacer - 1_2 Hex (217-2758):12
- [Angle] (0 deg): 1_2” Hex Bore Plastic VersaHub v2 (217-8079):5 ↔ 1_4 Acetal Spacer - 1_2 Hex (217-2758):12
- [Mate]: 1_2” Hex Bore Plastic VersaHub v2 (217-8079):5 ↔ 1_4 Acetal Spacer - 1_2 Hex (217-2758):12
- [Angle] (0 deg): 24T x 9mm Wide Double Flange Aluminum Pulley (HTD 5mm, 1_2” Hex Bore) (217-3227):5 ↔ 1_4 Acetal Spacer - 1_2 Hex (217-2758):12
- [Mate]: 24T x 9mm Wide Double Flange Aluminum Pulley (HTD 5mm, 1_2” Hex Bore) (217-3227):5 ↔ 1_4 Acetal Spacer - 1_2 Hex (217-2758):12
- [Angle] (0 deg): 1_2” Hex Bore Plastic VersaHub v2 (217-8079):6 ↔ 1_4 Acetal Spacer - 1_2 Hex (217-2758):11
- [Mate]: 1_2” Hex Bore Plastic VersaHub v2 (217-8079):6 ↔ 1_4 Acetal Spacer - 1_2 Hex (217-2758):11
- [Mate]: 1_2” Hex Bore Plastic VersaHub v2 (217-8079):6 ↔ 1_4 Acetal Spacer - 1_2 Hex (217-2758):11
- [Mate]: 1_4 Acetal Spacer - 1_2 Hex (217-2758):11 ↔ 24T x 9mm Wide Double Flange Aluminum Pulley (HTD 5mm, 1_2” Hex Bore) (217-3227):6
- [Angle] (0 deg): 1_4 Acetal Spacer - 1_2 Hex (217-2758):11 ↔ 24T x 9mm Wide Double Flange Aluminum Pulley (HTD 5mm, 1_2” Hex Bore) (217-3227):6
- [Mate]: 1_4 Acetal Spacer - 1_2 Hex (217-2758):11 ↔ 24T x 9mm Wide Double Flange Aluminum Pulley (HTD 5mm, 1_2” Hex Bore) (217-3227):6
- [Mate]: 5 Straight Flex Wheel (60A) (217-6455):5 ↔ 1_2” Hex Bore Plastic VersaHub v2 (217-8079):8
- [Mate]: 5 Straight Flex Wheel (60A) (217-6455):5 ↔ 1_2” Hex Bore Plastic VersaHub v2 (217-8079):8
- [Mate]: 5 Straight Flex Wheel (60A) (217-6455):5 ↔ 1_2” Hex Bore Plastic VersaHub v2 (217-8079):8
- [Mate]: 5 Straight Flex Wheel (60A) (217-6455):5 ↔ 1_2” Hex Bore Plastic VersaHub v2 (217-8079):7
- [Mate]: 5 Straight Flex Wheel (60A) (217-6455):5 ↔ 1_2” Hex Bore Plastic VersaHub v2 (217-8079):7
- [Mate]: 5 Straight Flex Wheel (60A) (217-6455):5 ↔ 1_2” Hex Bore Plastic VersaHub v2 (217-8079):7
- [Mate]: 1_2” Hex Bore Plastic VersaHub v2 (217-8079):7 ↔ #8-32 x 2.000 Star Drive Screw (276-8015):72
- [Mate]: 1_2” Hex Bore Plastic VersaHub v2 (217-8079):7 ↔ #8-32 x 2.000 Star Drive Screw (276-8015):71
- [Mate]: 1_2” Hex Bore Plastic VersaHub v2 (217-8079):7 ↔ #8-32 x 2.000 Star Drive Screw (276-8015):70
- [Mate]: 1_2” Hex Bore Plastic VersaHub v2 (217-8079):7 ↔ #8-32 x 2.000 Star Drive Screw (276-8015):69
- [Mate]: 1_2” Hex Bore Plastic VersaHub v2 (217-8079):7 ↔ #8-32 x 2.000 Star Drive Screw (276-8015):68
- [Mate]: 1_2” Hex Bore Plastic VersaHub v2 (217-8079):7 ↔ #8-32 x 2.000 Star Drive Screw (276-8015):67
- [Mate]: 1_2” Hex Bore Plastic VersaHub v2 (217-8079):7 ↔ #8-32 x 2.000 Star Drive Screw (276-8015):68
- [Mate]: 1_2” Hex Bore Plastic VersaHub v2 (217-8079):7 ↔ #8-32 x 2.000 Star Drive Screw (276-8015):71
- [Mate]: 1_2” Hex Bore Plastic VersaHub v2 (217-8079):7 ↔ #8-32 x 2.000 Star Drive Screw (276-8015):72
- [Mate]: 1_2” Hex Bore Plastic VersaHub v2 (217-8079):7 ↔ #8-32 x 2.000 Star Drive Screw (276-8015):67
- [Mate]: 1_2” Hex Bore Plastic VersaHub v2 (217-8079):7 ↔ #8-32 x 2.000 Star Drive Screw (276-8015):69
- [Mate]: 1_2” Hex Bore Plastic VersaHub v2 (217-8079):7 ↔ #8-32 x 2.000 Star Drive Screw (276-8015):70
- [Mate]: 1_2” Hex Bore Plastic VersaHub v2 (217-8079):7 ↔ 1_2 Acetal Spacer - 1_2 Hex (217-2758):4
- [Angle] (0 deg): 1_2” Hex Bore Plastic VersaHub v2 (217-8079):7 ↔ 1_2 Acetal Spacer - 1_2 Hex (217-2758):4
- [Mate]: 1_2” Hex Bore Plastic VersaHub v2 (217-8079):7 ↔ 1_2 Acetal Spacer - 1_2 Hex (217-2758):4
- [Angle] (0 deg): 1_2” Hex Bore Plastic VersaHub v2 (217-8079):8 ↔ 1_4 Acetal Spacer - 1_2 Hex (217-2758):8
- [Mate]: 1_2” Hex Bore Plastic VersaHub v2 (217-8079):8 ↔ 1_4 Acetal Spacer - 1_2 Hex (217-2758):8
- [Mate]: 1_2” Hex Bore Plastic VersaHub v2 (217-8079):8 ↔ 1_4 Acetal Spacer - 1_2 Hex (217-2758):8
- [Mate]: 1_4 Acetal Spacer - 1_2 Hex (217-2758):8 ↔ 24T x 9mm Wide Double Flange Aluminum Pulley (HTD 5mm, 1_2” Hex Bore) (217-3227):8
- [Angle] (0 deg): 1_4 Acetal Spacer - 1_2 Hex (217-2758):8 ↔ 24T x 9mm Wide Double Flange Aluminum Pulley (HTD 5mm, 1_2” Hex Bore) (217-3227):8
- [Mate]: 1_4 Acetal Spacer - 1_2 Hex (217-2758):8 ↔ 24T x 9mm Wide Double Flange Aluminum Pulley (HTD 5mm, 1_2” Hex Bore) (217-3227):8
- [Mate]: 5 Straight Flex Wheel (60A) (217-6455):6 ↔ 1_2” Hex Bore Plastic VersaHub v2 (217-8079):10
- [Mate]: 5 Straight Flex Wheel (60A) (217-6455):6 ↔ 1_2” Hex Bore Plastic VersaHub v2 (217-8079):10
- [Mate]: 5 Straight Flex Wheel (60A) (217-6455):6 ↔ 1_2” Hex Bore Plastic VersaHub v2 (217-8079):10
- [Mate]: 5 Straight Flex Wheel (60A) (217-6455):6 ↔ 1_2” Hex Bore Plastic VersaHub v2 (217-8079):9
- [Mate]: 5 Straight Flex Wheel (60A) (217-6455):6 ↔ 1_2” Hex Bore Plastic VersaHub v2 (217-8079):9
- [Mate]: 5 Straight Flex Wheel (60A) (217-6455):6 ↔ 1_2” Hex Bore Plastic VersaHub v2 (217-8079):9
- [Mate]: 1_2” Hex Bore Plastic VersaHub v2 (217-8079):9 ↔ #8-32 x 2.000 Star Drive Screw (276-8015):21
- [Mate]: 1_2” Hex Bore Plastic VersaHub v2 (217-8079):9 ↔ #8-32 x 2.000 Star Drive Screw (276-8015):22
- [Mate]: 1_2” Hex Bore Plastic VersaHub v2 (217-8079):9 ↔ #8-32 x 2.000 Star Drive Screw (276-8015):24
- [Mate]: 1_2” Hex Bore Plastic VersaHub v2 (217-8079):9 ↔ #8-32 x 2.000 Star Drive Screw (276-8015):19
- [Mate]: 1_2” Hex Bore Plastic VersaHub v2 (217-8079):9 ↔ #8-32 x 2.000 Star Drive Screw (276-8015):20
- [Mate]: 1_2” Hex Bore Plastic VersaHub v2 (217-8079):9 ↔ #8-32 x 2.000 Star Drive Screw (276-8015):23
- [Mate]: 1_2” Hex Bore Plastic VersaHub v2 (217-8079):9 ↔ #8-32 x 2.000 Star Drive Screw (276-8015):20
- [Mate]: 1_2” Hex Bore Plastic VersaHub v2 (217-8079):9 ↔ #8-32 x 2.000 Star Drive Screw (276-8015):22
- [Mate]: 1_2” Hex Bore Plastic VersaHub v2 (217-8079):9 ↔ #8-32 x 2.000 Star Drive Screw (276-8015):21
- [Mate]: 1_2” Hex Bore Plastic VersaHub v2 (217-8079):9 ↔ #8-32 x 2.000 Star Drive Screw (276-8015):23
- [Mate]: 1_2” Hex Bore Plastic VersaHub v2 (217-8079):9 ↔ #8-32 x 2.000 Star Drive Screw (276-8015):19
- [Mate]: 1_2” Hex Bore Plastic VersaHub v2 (217-8079):9 ↔ #8-32 x 2.000 Star Drive Screw (276-8015):24
- [Mate]: #8-32 x 2.000 Star Drive Screw (276-8015):21 ↔ #8-32 Nylock Nut (275-1027):24
- [Mate]: #8-32 x 2.000 Star Drive Screw (276-8015):24 ↔ #8-32 Nylock Nut (275-1027):19
- [Mate]: #8-32 x 2.000 Star Drive Screw (276-8015):19 ↔ #8-32 Nylock Nut (275-1027):23
- [Mate]: #8-32 x 2.000 Star Drive Screw (276-8015):23 ↔ #8-32 Nylock Nut (275-1027):20
- [Mate]: #8-32 x 2.000 Star Drive Screw (276-8015):20 ↔ #8-32 Nylock Nut (275-1027):22
- [Mate]: #8-32 x 2.000 Star Drive Screw (276-8015):22 ↔ #8-32 Nylock Nut (275-1027):21
- [Mate]: 1_2” Hex Bore Plastic VersaHub v2 (217-8079):10 ↔ #8-32 Nylock Nut (275-1027):24
- [Mate]: 1_2” Hex Bore Plastic VersaHub v2 (217-8079):10 ↔ #8-32 Nylock Nut (275-1027):21
- [Mate]: 1_2” Hex Bore Plastic VersaHub v2 (217-8079):10 ↔ #8-32 Nylock Nut (275-1027):22
- [Mate]: 1_2” Hex Bore Plastic VersaHub v2 (217-8079):10 ↔ #8-32 Nylock Nut (275-1027):20
- [Mate]: 1_2” Hex Bore Plastic VersaHub v2 (217-8079):10 ↔ #8-32 Nylock Nut (275-1027):23
- [Mate]: 1_2” Hex Bore Plastic VersaHub v2 (217-8079):10 ↔ #8-32 Nylock Nut (275-1027):19
- [Angle] (0 deg): 1_2” Hex Bore Plastic VersaHub v2 (217-8079):10 ↔ #8-32 Nylock Nut (275-1027):24
- [Angle] (0 deg): 1_2” Hex Bore Plastic VersaHub v2 (217-8079):10 ↔ #8-32 Nylock Nut (275-1027):19
- [Angle] (0 deg): 1_2” Hex Bore Plastic VersaHub v2 (217-8079):10 ↔ #8-32 Nylock Nut (275-1027):23
- [Angle] (0 deg): 1_2” Hex Bore Plastic VersaHub v2 (217-8079):10 ↔ #8-32 Nylock Nut (275-1027):20
- [Angle] (0 deg): 1_2” Hex Bore Plastic VersaHub v2 (217-8079):10 ↔ #8-32 Nylock Nut (275-1027):22
- [Angle] (0 deg): 1_2” Hex Bore Plastic VersaHub v2 (217-8079):10 ↔ #8-32 Nylock Nut (275-1027):21
- [Mate]: 1_2” Hex Bore Plastic VersaHub v2 (217-8079):9 ↔ 1_4 Acetal Spacer - 1_2 Hex (217-2758):9
- [Angle] (0 deg): 1_2” Hex Bore Plastic VersaHub v2 (217-8079):9 ↔ 1_4 Acetal Spacer - 1_2 Hex (217-2758):9
- [Mate]: 1_2” Hex Bore Plastic VersaHub v2 (217-8079):9 ↔ 1_4 Acetal Spacer - 1_2 Hex (217-2758):9
- [Mate]: 5 Straight Flex Wheel (60A) (217-6455):10 ↔ 1_2” Hex Bore Plastic VersaHub v2 (217-8079):18
- [Mate]: 5 Straight Flex Wheel (60A) (217-6455):10 ↔ 1_2” Hex Bore Plastic VersaHub v2 (217-8079):18
- [Mate]: 5 Straight Flex Wheel (60A) (217-6455):10 ↔ 1_2” Hex Bore Plastic VersaHub v2 (217-8079):18
- [Mate]: 5 Straight Flex Wheel (60A) (217-6455):10 ↔ 1_2” Hex Bore Plastic VersaHub v2 (217-8079):17
- [Mate]: 5 Straight Flex Wheel (60A) (217-6455):10 ↔ 1_2” Hex Bore Plastic VersaHub v2 (217-8079):17
- [Mate]: 5 Straight Flex Wheel (60A) (217-6455):10 ↔ 1_2” Hex Bore Plastic VersaHub v2 (217-8079):17
- [Mate]: 1_2” Hex Bore Plastic VersaHub v2 (217-8079):17 ↔ #8-32 x 2.000 Star Drive Screw (276-8015):45
- [Mate]: 1_2” Hex Bore Plastic VersaHub v2 (217-8079):17 ↔ #8-32 x 2.000 Star Drive Screw (276-8015):46
- Mate:346: 1_2” Hex Bore Plastic VersaHub v2 (217-8079):17 ↔ #8-32 x 2.000 Star Drive Screw (276-8015):48
- Mate:347: 1_2” Hex Bore Plastic VersaHub v2 (217-8079):17 ↔ #8-32 x 2.000 Star Drive Screw (276-8015):43
- [Mate]: 1_2” Hex Bore Plastic VersaHub v2 (217-8079):17 ↔ #8-32 x 2.000 Star Drive Screw (276-8015):44
- [Mate]: 1_2” Hex Bore Plastic VersaHub v2 (217-8079):17 ↔ #8-32 x 2.000 Star Drive Screw (276-8015):47
- [Mate]: 1_2” Hex Bore Plastic VersaHub v2 (217-8079):17 ↔ #8-32 x 2.000 Star Drive Screw (276-8015):44
- [Mate]: 1_2” Hex Bore Plastic VersaHub v2 (217-8079):17 ↔ #8-32 x 2.000 Star Drive Screw (276-8015):46
- [Mate]: 1_2” Hex Bore Plastic VersaHub v2 (217-8079):17 ↔ #8-32 x 2.000 Star Drive Screw (276-8015):45
- [Mate]: 1_2” Hex Bore Plastic VersaHub v2 (217-8079):17 ↔ #8-32 x 2.000 Star Drive Screw (276-8015):47
- [Mate]: 1_2” Hex Bore Plastic VersaHub v2 (217-8079):17 ↔ #8-32 x 2.000 Star Drive Screw (276-8015):43
- [Mate]: 1_2” Hex Bore Plastic VersaHub v2 (217-8079):17 ↔ #8-32 x 2.000 Star Drive Screw (276-8015):48
- [Mate]: #8-32 x 2.000 Star Drive Screw (276-8015):45 ↔ #8-32 Nylock Nut (275-1027):48
- [Mate]: #8-32 x 2.000 Star Drive Screw (276-8015):48 ↔ #8-32 Nylock Nut (275-1027):43
- [Mate]: #8-32 x 2.000 Star Drive Screw (276-8015):43 ↔ #8-32 Nylock Nut (275-1027):47
- [Mate]: #8-32 x 2.000 Star Drive Screw (276-8015):47 ↔ #8-32 Nylock Nut (275-1027):44
- [Mate]: #8-32 x 2.000 Star Drive Screw (276-8015):44 ↔ #8-32 Nylock Nut (275-1027):46
- [Mate]: #8-32 x 2.000 Star Drive Screw (276-8015):46 ↔ #8-32 Nylock Nut (275-1027):45
- [Mate]: 1_2” Hex Bore Plastic VersaHub v2 (217-8079):18 ↔ #8-32 Nylock Nut (275-1027):48
- [Mate]: 1_2” Hex Bore Plastic VersaHub v2 (217-8079):18 ↔ #8-32 Nylock Nut (275-1027):45
- [Mate]: 1_2” Hex Bore Plastic VersaHub v2 (217-8079):18 ↔ #8-32 Nylock Nut (275-1027):46
- [Mate]: 1_2” Hex Bore Plastic VersaHub v2 (217-8079):18 ↔ #8-32 Nylock Nut (275-1027):44
- [Mate]: 1_2” Hex Bore Plastic VersaHub v2 (217-8079):18 ↔ #8-32 Nylock Nut (275-1027):47
- [Mate]: 1_2” Hex Bore Plastic VersaHub v2 (217-8079):18 ↔ #8-32 Nylock Nut (275-1027):43
- [Angle] (0 deg): 1_2” Hex Bore Plastic VersaHub v2 (217-8079):18 ↔ #8-32 Nylock Nut (275-1027):48
- [Angle] (0 deg): 1_2” Hex Bore Plastic VersaHub v2 (217-8079):18 ↔ #8-32 Nylock Nut (275-1027):43
- [Angle] (0 deg): 1_2” Hex Bore Plastic VersaHub v2 (217-8079):18 ↔ #8-32 Nylock Nut (275-1027):47
- [Angle] (0 deg): 1_2” Hex Bore Plastic VersaHub v2 (217-8079):18 ↔ #8-32 Nylock Nut (275-1027):44
- [Angle] (0 deg): 1_2” Hex Bore Plastic VersaHub v2 (217-8079):18 ↔ #8-32 Nylock Nut (275-1027):46
- [Angle] (0 deg): 1_2” Hex Bore Plastic VersaHub v2 (217-8079):18 ↔ #8-32 Nylock Nut (275-1027):45
- [Angle] (0 deg): 1_2” Hex Bore Plastic VersaHub v2 (217-8079):18 ↔ 1_4 Acetal Spacer - 1_2 Hex (217-2758):13
- [Mate]: 1_2” Hex Bore Plastic VersaHub v2 (217-8079):18 ↔ 1_4 Acetal Spacer - 1_2 Hex (217-2758):13
- [Mate]: 5 Straight Flex Wheel (60A) (217-6455):11 ↔ 1_2” Hex Bore Plastic VersaHub v2 (217-8079):20
- [Mate]: 5 Straight Flex Wheel (60A) (217-6455):11 ↔ 1_2” Hex Bore Plastic VersaHub v2 (217-8079):20
- [Mate]: 5 Straight Flex Wheel (60A) (217-6455):11 ↔ 1_2” Hex Bore Plastic VersaHub v2 (217-8079):20
- [Mate]: 5 Straight Flex Wheel (60A) (217-6455):11 ↔ 1_2” Hex Bore Plastic VersaHub v2 (217-8079):19
- [Mate]: 5 Straight Flex Wheel (60A) (217-6455):11 ↔ 1_2” Hex Bore Plastic VersaHub v2 (217-8079):19
- [Mate]: 5 Straight Flex Wheel (60A) (217-6455):11 ↔ 1_2” Hex Bore Plastic VersaHub v2 (217-8079):19
- [Mate]: 1_2” Hex Bore Plastic VersaHub v2 (217-8079):19 ↔ #8-32 x 2.000 Star Drive Screw (276-8015):51
- [Mate]: 1_2” Hex Bore Plastic VersaHub v2 (217-8079):19 ↔ #8-32 x 2.000 Star Drive Screw (276-8015):52
- [Mate]: 1_2” Hex Bore Plastic VersaHub v2 (217-8079):19 ↔ #8-32 x 2.000 Star Drive Screw (276-8015):54
- [Mate]: 1_2” Hex Bore Plastic VersaHub v2 (217-8079):19 ↔ #8-32 x 2.000 Star Drive Screw (276-8015):49
- [Mate]: 1_2” Hex Bore Plastic VersaHub v2 (217-8079):19 ↔ #8-32 x 2.000 Star Drive Screw (276-8015):50
- [Mate]: 1_2” Hex Bore Plastic VersaHub v2 (217-8079):19 ↔ #8-32 x 2.000 Star Drive Screw (276-8015):53
- [Mate]: 1_2” Hex Bore Plastic VersaHub v2 (217-8079):19 ↔ #8-32 x 2.000 Star Drive Screw (276-8015):50
- [Mate]: 1_2” Hex Bore Plastic VersaHub v2 (217-8079):19 ↔ #8-32 x 2.000 Star Drive Screw (276-8015):52
- [Mate]: 1_2” Hex Bore Plastic VersaHub v2 (217-8079):19 ↔ #8-32 x 2.000 Star Drive Screw (276-8015):51
- [Mate]: 1_2” Hex Bore Plastic VersaHub v2 (217-8079):19 ↔ #8-32 x 2.000 Star Drive Screw (276-8015):53
- [Mate]: 1_2” Hex Bore Plastic VersaHub v2 (217-8079):19 ↔ #8-32 x 2.000 Star Drive Screw (276-8015):49
- [Mate]: 1_2” Hex Bore Plastic VersaHub v2 (217-8079):19 ↔ #8-32 x 2.000 Star Drive Screw (276-8015):54
- [Mate]: #8-32 x 2.000 Star Drive Screw (276-8015):51 ↔ #8-32 Nylock Nut (275-1027):54
- [Mate]: #8-32 x 2.000 Star Drive Screw (276-8015):54 ↔ #8-32 Nylock Nut (275-1027):49
- [Mate]: #8-32 x 2.000 Star Drive Screw (276-8015):49 ↔ #8-32 Nylock Nut (275-1027):53
- [Mate]: #8-32 x 2.000 Star Drive Screw (276-8015):53 ↔ #8-32 Nylock Nut (275-1027):50
- [Mate]: #8-32 x 2.000 Star Drive Screw (276-8015):50 ↔ #8-32 Nylock Nut (275-1027):52
- [Mate]: #8-32 x 2.000 Star Drive Screw (276-8015):52 ↔ #8-32 Nylock Nut (275-1027):51
- [Mate]: 1_2” Hex Bore Plastic VersaHub v2 (217-8079):20 ↔ #8-32 Nylock Nut (275-1027):54
- [Mate]: 1_2” Hex Bore Plastic VersaHub v2 (217-8079):20 ↔ #8-32 Nylock Nut (275-1027):51
- [Mate]: 1_2” Hex Bore Plastic VersaHub v2 (217-8079):20 ↔ #8-32 Nylock Nut (275-1027):52
- [Mate]: 1_2” Hex Bore Plastic VersaHub v2 (217-8079):20 ↔ #8-32 Nylock Nut (275-1027):50
- [Mate]: 1_2” Hex Bore Plastic VersaHub v2 (217-8079):20 ↔ #8-32 Nylock Nut (275-1027):53